# Autodesk Inventor assembly: Bearing with Screw Generator
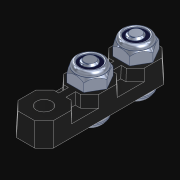
[picture p0: Inventor's stored thumbnail of the model, 180x180]
Saved by Autodesk Inventor 2021.3 (Build 253353010, 353A)
## iProperties
Created: 2021-07-20
Part Number: Bearing with Screw Generator
Document SubType Name: Assembly
Designer: yuany
Author: yuany
## Documents named in this file (15)
- E:\VEX Cad\Inventor Library\Motion\Bearings with Screws\Bearing with Screw Generator.iam
- E:\VEX Cad\Inventor Library\Motion\Bearing Flat.ipt
- E:\VEX Cad\Inventor Library\Structure\Hardware\Nut Alu.ipt
- E:\VEX Cad\Inventor Library\Structure\Hardware\Nut Hex.ipt
- E:\VEX Cad\Inventor Library\Structure\Hardware\Nut Keps.ipt
- E:\VEX Cad\Inventor Library\Structure\Hardware\Nut Nylock.ipt
- E:\VEX Cad\Inventor Library\Structure\Hardware\Nut Nylon - Black.ipt
- E:\VEX Cad\Inventor Library\Structure\Hardware\Nut Nylon - White.ipt
- E:\VEX Cad\Inventor Library\Structure\Hardware\Nut Thin Nylock.ipt
- E:\VEX Cad\Inventor Library\Structure\Hardware\Screw Alu\AScrew .500 Threaded.ipt
- E:\VEX Cad\Inventor Library\Structure\Hardware\Screw Alu.ipt
- E:\VEX Cad\Inventor Library\Structure\Hardware\Screw Steel - Star\Screw 8-32 Steel .500 Threaded.ipt
- E:\VEX Cad\Inventor Library\Structure\Hardware\Screw Steel - Star.ipt
- E:\VEX Cad\Inventor Library\Structure\Hardware\Screw Steel - Hex\Screw 8-32 Steel .500 Threaded.ipt
- E:\VEX Cad\Inventor Library\Structure\Hardware\Screw Steel - Hex.ipt
## Components (31 placed, 10 different names)
1. Bearing Flat:1 — Insert:1, Insert:2, Insert:3, Insert:4, Insert:5, Insert:6, Insert:7, Insert:8, Insert:9, Insert:10, Insert:11, Insert:12, Insert:13, Insert:14, Insert:15, Insert:16, Insert:17, Insert:18, Insert:19, Insert:20, Insert:21, Insert:22, Insert:23, Insert:24, Insert:25, Insert:26, Insert:27, Insert:28, Insert:29, Insert:30
2. Nut Alu:1 — Insert:1
3. Nut Alu:2 — Insert:2
4. Nut Alu:3 — Insert:3
5. Nut Keps:1 — Insert:18
6. Nut Keps:2 — Insert:17
7. Nut Keps:3 — Insert:16
8. Nut Nylock:1 — Insert:15
9. Nut Nylock:2 — Insert:14
10. Nut Nylock:3 — Insert:13
11. Nut Nylon - Black:1 — Insert:7
12. Nut Nylon - Black:2 — Insert:8
13. Nut Nylon - Black:3 — Insert:9
14. Nut Nylon - White:1 — Insert:4
15. Nut Nylon - White:2 — Insert:5
16. Nut Nylon - White:3 — Insert:6
17. Nut Thin Nylock:1 — Insert:11
18. Nut Thin Nylock:2 — Insert:12
19. Nut Thin Nylock:3 — Insert:10
20. Nut Hex:1 — Insert:21
21. Nut Hex:2 — Insert:20
22. Nut Hex:3 — Insert:19
23. AScrew .500 Threaded:1 — Insert:25
24. AScrew .500 Threaded:2 — Insert:26
25. AScrew .500 Threaded:3 — Insert:27
26. Screw 8-32 Steel .500 Threaded:1 — Insert:22
27. Screw 8-32 Steel .500 Threaded:2 — Insert:23
28. Screw 8-32 Steel .500 Threaded:3 — Insert:24
29. Screw 8-32 Steel .500 Threaded:1 — Insert:29
30. Screw 8-32 Steel .500 Threaded:2 — Insert:30
31. Screw 8-32 Steel .500 Threaded:3 — Insert:28
## Relationships (30: Insert 30)
- Insert:1: Bearing Flat:1 ↔ Nut Alu:1
- Insert:2: Bearing Flat:1 ↔ Nut Alu:2
- Insert:3: Bearing Flat:1 ↔ Nut Alu:3
- Insert:4: Bearing Flat:1 ↔ Nut Nylon - White:1
- Insert:5: Bearing Flat:1 ↔ Nut Nylon - White:2
- Insert:6: Bearing Flat:1 ↔ Nut Nylon - White:3
- Insert:7: Bearing Flat:1 ↔ Nut Nylon - Black:1
- Insert:8: Bearing Flat:1 ↔ Nut Nylon - Black:2
- Insert:9: Bearing Flat:1 ↔ Nut Nylon - Black:3
- Insert:10: Bearing Flat:1 ↔ Nut Thin Nylock:3
- Insert:11: Bearing Flat:1 ↔ Nut Thin Nylock:1
- Insert:12: Bearing Flat:1 ↔ Nut Thin Nylock:2
- Insert:13: Bearing Flat:1 ↔ Nut Nylock:3
- Insert:14: Bearing Flat:1 ↔ Nut Nylock:2
- Insert:15: Bearing Flat:1 ↔ Nut Nylock:1
- Insert:16: Bearing Flat:1 ↔ Nut Keps:3
- Insert:17: Bearing Flat:1 ↔ Nut Keps:2
- Insert:18: Bearing Flat:1 ↔ Nut Keps:1
- Insert:19: Bearing Flat:1 ↔ Nut Hex:3
- Insert:20: Bearing Flat:1 ↔ Nut Hex:2
- Insert:21: Bearing Flat:1 ↔ Nut Hex:1
- Insert:22 (1.6002 mm): Bearing Flat:1 ↔ Screw 8-32 Steel .500 Threaded:1
- Insert:23 (1.6002 mm): Bearing Flat:1 ↔ Screw 8-32 Steel .500 Threaded:2
- Insert:24 (1.6002 mm): Bearing Flat:1 ↔ Screw 8-32 Steel .500 Threaded:3
- Insert:25 (1.6002 mm): Bearing Flat:1 ↔ AScrew .500 Threaded:1
- Insert:26 (1.6002 mm): Bearing Flat:1 ↔ AScrew .500 Threaded:2
- Insert:27 (1.6002 mm): Bearing Flat:1 ↔ AScrew .500 Threaded:3
- Insert:28 (1.6002 mm): Bearing Flat:1 ↔ Screw 8-32 Steel .500 Threaded:3
- Insert:29 (1.6002 mm): Bearing Flat:1 ↔ Screw 8-32 Steel .500 Threaded:1
- Insert:30 (1.6002 mm): Bearing Flat:1 ↔ Screw 8-32 Steel .500 Threaded:2
## Named parameters: Metal = 1.6002 mm
